# Autodesk Inventor assembly: herkulex assembled
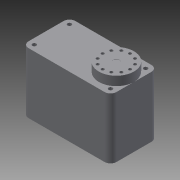
[picture p0: Inventor's stored thumbnail of the model, 180x180]
Saved by Autodesk Inventor 2015 (Build 190159000, 159)
## iProperties
Created: 2014-10-18
Part Number: herkulex assembled
Document SubType Name: Assembly
Designer: ericd_000
Author: ericd_000
## Documents named in this file (4)
- C:\Users\ericd_000\Dropbox\GitHub\initial_cad\eric_cad\herkulex assembled.iam
- C:\Users\ericd_000\Dropbox\GitHub\initial_cad\eric_cad\herkulex pin.ipt
- C:\Users\ericd_000\Dropbox\GitHub\initial_cad\eric_cad\herkulex spinner.ipt
- C:\Users\ericd_000\Dropbox\GitHub\initial_cad\eric_cad\herkulex.ipt
## Components (3 placed, 3 different names)
1. herkulex pin:1 — Cylindrical:1, Rotational:3, Flush:1
2. herkulex spinner:1 — Rotational:3, Mate:1, Flush:1
3. herkulex:1 — Cylindrical:1, Mate:1
## Relationships (4: CylindricalJoint 1, RevoluteJoint 1, Mate 1, Flush 1)
- Cylindrical:1: herkulex pin:1 ↔ herkulex:1
- Rotational:3 [RevoluteJoint]: herkulex pin:1 ↔ herkulex spinner:1
- Mate:1: herkulex spinner:1 ↔ herkulex:1
- Flush:1: herkulex pin:1 ↔ herkulex spinner:1
